# Autodesk Inventor assembly: assembly_holder2
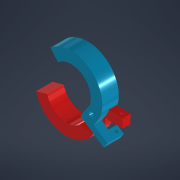
[picture p0: Inventor's stored thumbnail of the model, 180x180]
Saved by Autodesk Inventor 2021 (Build 250183000, 183)
## iProperties
Created: 2021-06-04
Part Number: assembly_holder2
Document SubType Name: Assembly
Designer: Watchdog
Author: Watchdog
## Documents named in this file (3)
- C:\Users\Watchdog\OneDrive - Flinders\Advn Mech Design Shared\6_Development\2_Design\inventor\securing_mechanism\securingMechanism_variant_vertical_x\assembly_holder2.iam
- C:\Users\Watchdog\OneDrive - Flinders\Advn Mech Design Shared\6_Development\2_Design\inventor\securing_mechanism\securingMechanism_variant_vertical_x\holder2_base.ipt
- C:\Users\Watchdog\OneDrive - Flinders\Advn Mech Design Shared\6_Development\2_Design\inventor\securing_mechanism\securingMechanism_variant_vertical_x\holder2_clamp.ipt
## Components (2 placed, 2 different names)
1. holder2_base:1 — Flush:1, Mate:2, Mate:3, Flush:2
2. holder2_clamp:1 — Mate:3, Flush:2
## Relationships (4: Flush 2, Mate 2)
- Flush:1: holder2_base:1
- Mate:2: holder2_base:1
- Mate:3: holder2_base:1 ↔ holder2_clamp:1
- Flush:2: holder2_base:1 ↔ holder2_clamp:1
